# Autodesk Inventor assembly: SnowBlowerMotorMountAndHub
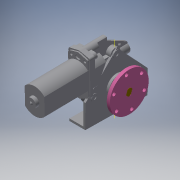
[picture p0: Inventor's stored thumbnail of the model, 180x180]
Saved by Autodesk Inventor 2016 SP1 (Build 200210100, 210)
## iProperties
Created: 2016-02-07
Part Number: SnowBlowerMotorMountAndHub
Document SubType Name: Assembly
Designer: steele
Author: steele
## Documents named in this file (3)
- C:\snobotics\CAD-Development\robSteele\SnoBotics2016\AM Parts\SnowBlowerMotorMountAndHub.iam
- C:\snobotics\CAD-Development\robSteele\SnoBotics2016\AM Parts\SnowBlowerMotorAndHub.iam
- C:\snobotics\CAD-Development\robSteele\SnoBotics2016\AM Parts\rsSnowBlowerMount.ipt
## Components (2 placed, 2 different names)
1. rsSnowBlowerMount:1 — Insert:1
2. SnowBlowerMotorAndHub:1 [sub-assembly] — Insert:1
## Relationships (1: Insert 1)
- Insert:1: rsSnowBlowerMount:1 ↔ SnowBlowerMotorAndHub:1
